# Autodesk Inventor assembly: ASY GBK короткая стенка
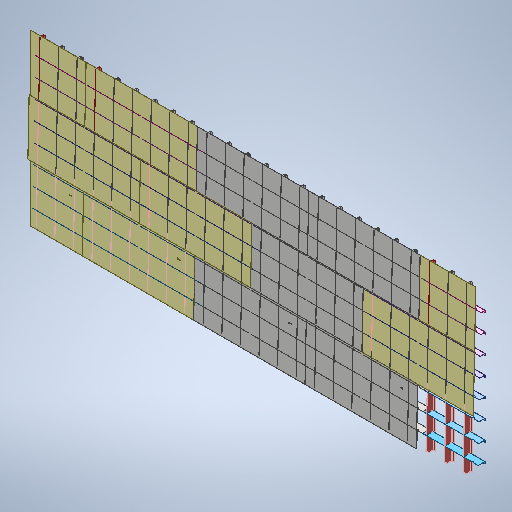
[picture p0: Inventor's stored thumbnail of the model, 512x512]
Saved by Autodesk Inventor 2026.2 (Build 302298000, 298)
## iProperties
Created: 2026-05-24
Part Number: ASY GBK короткая стенка
Document SubType Name: Assembly
Designer: pokla
Author: pokla
## Documents named in this file (10)
- C:\Users\admin\Documents\Inventor\GBK-Gubkinskiy\ASY GBK короткая стенка.iam
- C:\Users\admin\Documents\Inventor\GBK-Gubkinskiy\ASY GBK 2110 short wall shield 1.iam
- C:\Users\admin\Documents\Inventor\GBK-Gubkinskiy\ASY GBK 2120 short wall shield 2.iam
- C:\Users\admin\Documents\Inventor\GBK-Gubkinskiy\ASY GBK 2130 short wall shield 3.iam
- C:\Users\admin\Documents\Inventor\GBK-Gubkinskiy\ASY GBK 2210 short wall shield 4.iam
- C:\Users\admin\Documents\Inventor\GBK-Gubkinskiy\ASY GBK 2310 short wall shield 7.iam
- C:\Users\admin\Documents\Inventor\GBK-Gubkinskiy\ASY GBK 2320 short wall shield 8.iam
- C:\Users\admin\Documents\Inventor\GBK-Gubkinskiy\ASY GBK 2330 short wall shield 9.iam
- C:\Users\admin\Documents\Inventor\GBK-Gubkinskiy\ASY GBK 2220 short wall shield 5.iam
- C:\Users\admin\Documents\Inventor\GBK-Gubkinskiy\ASY GBK 2230 short wall shield 6.iam
## Components (14 placed, 9 different names)
1. ASY GBK 2110 short wall shield 1.iam:1 [sub-assembly] — Rigid:1, Rigid:5
2. ASY GBK 2120 short wall shield 2.iam:1 [sub-assembly] — Rigid:1, Rigid:2
3. ASY GBK 2120 short wall shield 2.iam:2 [sub-assembly] — Rigid:2, Rigid:3
4. ASY GBK 2120 short wall shield 2.iam:3 [sub-assembly] — Rigid:3, Rigid:4
5. ASY GBK 2130 short wall shield 3.iam:1 [sub-assembly] — Rigid:4
6. ASY GBK 2210 short wall shield 4.iam:1 [sub-assembly] — Rigid:5, Rigid:6, Rigid:9
7. ASY GBK 2220 short wall shield 5.iam:1 [sub-assembly] — Rigid:6, Rigid:7
8. ASY GBK 2220 short wall shield 5.iam:2 [sub-assembly] — Rigid:7, Rigid:8
9. ASY GBK 2230 short wall shield 6.iam:1 [sub-assembly] — Rigid:8
10. ASY GBK 2310 short wall shield 7.iam:1 [sub-assembly] — Rigid:9, Rigid:10
11. ASY GBK 2320 short wall shield 8.iam:1 [sub-assembly] — Rigid:10, Rigid:11
12. ASY GBK 2330 short wall shield 9.iam:1 [sub-assembly] — Rigid:13
13. ASY GBK 2320 short wall shield 8.iam:2 [sub-assembly] — Rigid:11, Rigid:12
14. ASY GBK 2320 short wall shield 8.iam:3 [sub-assembly] — Rigid:12, Rigid:13
## Relationships (13: WeldJoint 13)
- Rigid:1 [WeldJoint]: ASY GBK 2110 short wall shield 1.iam:1 ↔ ASY GBK 2120 short wall shield 2.iam:1
- Rigid:2 [WeldJoint]: ASY GBK 2120 short wall shield 2.iam:1 ↔ ASY GBK 2120 short wall shield 2.iam:2
- Rigid:3 [WeldJoint]: ASY GBK 2120 short wall shield 2.iam:2 ↔ ASY GBK 2120 short wall shield 2.iam:3
- Rigid:4 [WeldJoint]: ASY GBK 2120 short wall shield 2.iam:3 ↔ ASY GBK 2130 short wall shield 3.iam:1
- Rigid:5 [WeldJoint]: ASY GBK 2110 short wall shield 1.iam:1 ↔ ASY GBK 2210 short wall shield 4.iam:1
- Rigid:6 [WeldJoint]: ASY GBK 2210 short wall shield 4.iam:1 ↔ ASY GBK 2220 short wall shield 5.iam:1
- Rigid:7 [WeldJoint]: ASY GBK 2220 short wall shield 5.iam:1 ↔ ASY GBK 2220 short wall shield 5.iam:2
- Rigid:8 [WeldJoint]: ASY GBK 2220 short wall shield 5.iam:2 ↔ ASY GBK 2230 short wall shield 6.iam:1
- Rigid:9 [WeldJoint]: ASY GBK 2210 short wall shield 4.iam:1 ↔ ASY GBK 2310 short wall shield 7.iam:1
- Rigid:10 [WeldJoint]: ASY GBK 2310 short wall shield 7.iam:1 ↔ ASY GBK 2320 short wall shield 8.iam:1
- Rigid:11 [WeldJoint]: ASY GBK 2320 short wall shield 8.iam:1 ↔ ASY GBK 2320 short wall shield 8.iam:2
- Rigid:12 [WeldJoint]: ASY GBK 2320 short wall shield 8.iam:2 ↔ ASY GBK 2320 short wall shield 8.iam:3
- Rigid:13 [WeldJoint]: ASY GBK 2330 short wall shield 9.iam:1 ↔ ASY GBK 2320 short wall shield 8.iam:3
